# Autodesk Inventor assembly: Quad Cart
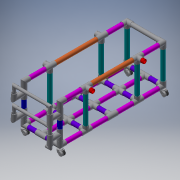
[picture p0: Inventor's stored thumbnail of the model, 180x180]
Saved by Autodesk Inventor 2018 (Build 220112000, 112)
## iProperties
Created: 2017-11-03
Part Number: Quad Cart
Document SubType Name: Assembly
Designer: owner
Author: owner
## Documents named in this file (29)
- Z:\The Pickle\Final Carts\Quad Cart.iam
- Z:\The Pickle\Inventor Pipe Parts\1.5 3-way 90.ipt
- Z:\The Pickle\Inventor Pipe Parts\Quad Pipes\1.5 pipe - 1.ipt
- Z:\The Pickle\Inventor Pipe Parts\Quad Pipes\1.5 pipe - 2.ipt
- Z:\The Pickle\Inventor Pipe Parts\1.5 Tee.ipt
- Z:\The Pickle\Inventor Pipe Parts\1.5 Tee 4-way.ipt
- Z:\The Pickle\Inventor Pipe Parts\Quad Pipes\1.5 pipe - 7.ipt
- Z:\The Pickle\Inventor Pipe Parts\Quad Pipes\1.5 pipe - 3.ipt
- Z:\The Pickle\Inventor Pipe Parts\1.5 cross.ipt
- Z:\The Pickle\Inventor Pipe Parts\Quad Pipes\1.5 pipe - 6.ipt
- Z:\The Pickle\Inventor Pipe Parts\1.5 90.ipt
- Z:\The Pickle\Inventor Pipe Parts\Quad Pipes\1.5 pipe - 4.ipt
- Z:\The Pickle\Inventor Pipe Parts\1.5 Tee 4-way_MIR.ipt
- Z:\The Pickle\Inventor Pipe Parts\Quad Pipes\1.5 pipe - 1_MIR.ipt
- Z:\The Pickle\Inventor Pipe Parts\Quad Pipes\1.5 pipe - 2_MIR.ipt
- Z:\The Pickle\Inventor Pipe Parts\Quad Pipes\1.5 pipe - 3_MIR.ipt
- Z:\The Pickle\Inventor Pipe Parts\1.5 Tee_MIR.ipt
- Z:\The Pickle\Inventor Pipe Parts\1.5 3-way 90_MIR.ipt
- Z:\The Pickle\Inventor Pipe Parts\Quad Pipes\1.5 pipe - 4_MIR.ipt
- Z:\The Pickle\Inventor Pipe Parts\Quad Pipes\1.5 pipe - 2_MIR_MIR.ipt
- Z:\The Pickle\Inventor Pipe Parts\Quad Pipes\1.5 pipe - 5.ipt
- Z:\The Pickle\Inventor Pipe Parts\Quad Pipes\1 pipe - 1.ipt
- Z:\The Pickle\Inventor Pipe Parts\Quad Pipes\1 pipe - 2.ipt
- Z:\The Pickle\Inventor Pipe Parts\Quad Pipes\1 pipe - 3.ipt
- Z:\The Pickle\Inventor Pipe Parts\Quad Pipes\1 pipe - 4.ipt
- Z:\The Pickle\Inventor Pipe Parts\1 90.ipt
- Z:\The Pickle\Inventor Pipe Parts\1 tee.ipt
- Z:\The Pickle\Inventor Pipe Parts\Wheel Part.ipt
- Z:\The Pickle\Inventor Pipe Parts\NUT.ipt
## Components (97 placed, 28 different names)
1. 1.5 3-way 90:1 — Insert:1, Insert:41, Insert:106, Insert:113, Flush:1, Insert:120
2. 1.5 pipe - 1:1 — Insert:41, Insert:42
3. 1.5 pipe - 2:1 — Insert:1, Insert:22
4. 1.5 Tee:2 — Insert:42, Insert:43, Insert:45
5. 1.5 Tee 4-way:1 — Insert:22, Insert:24, Insert:35, Insert:60
6. 1.5 Tee:3 — Insert:4, Insert:6, Insert:107
7. 1.5 pipe - 1:2 — Insert:43, Insert:44
8. 1.5 pipe - 1:3 — Insert:59, Insert:60
9. 1.5 pipe - 7:1 — Insert:6, Insert:7
10. 1.5 pipe - 2:2 — Insert:45, Insert:46
11. 1.5 pipe - 2:3 — Insert:24, Insert:27
12. 1.5 pipe - 3:1 — Insert:35, Insert:127
13. 1.5 3-way 90:2 — Insert:44, Insert:71, Insert:108, Insert:114, Insert:119
14. 1.5 Tee:4 — Insert:27, Insert:28, Insert:58
15. 1.5 Tee:5 — Insert:5
16. 1.5 Tee:6 — Insert:7, Insert:8, Insert:105
17. 1.5 cross:1 — Insert:46, Insert:47, Insert:59, Insert:61
18. 1.5 pipe - 6:1 — Insert:4, Insert:5
19. 1.5 pipe - 6:2 — Insert:8, Insert:9
20. 1.5 pipe - 6:3 — Insert:14, Insert:15
21. 1.5 pipe - 6:4 — Insert:18, Insert:19
22. 1.5 pipe - 7:2 — Insert:16, Insert:17
23. 1.5 Tee:8 — Insert:14, Insert:16, Insert:109
24. 1.5 Tee:9 — Insert:17, Insert:18, Insert:103
25. 1.5 90:1 — Insert:15
26. 1.5 90:2 — Insert:19
27. 1.5 90:3 — Insert:23, Insert:104
28. 1.5 Tee:10 — Insert:9, Insert:112
29. 1.5 90:4 — Insert:88, Insert:102
30. 1.5 cross:2 — Insert:48, Insert:49, Insert:57, Insert:62
31. 1.5 cross:3 — Insert:50, Insert:51, Insert:55, Insert:63
32. 1.5 Tee:11 — Insert:52, Insert:53, Insert:64
33. 1.5 pipe - 2:4 — Insert:47, Insert:48
34. 1.5 pipe - 2:5 — Insert:49, Insert:50
35. 1.5 pipe - 2:6 — Insert:51, Insert:52
36. 1.5 pipe - 2:7 — Insert:28, Insert:29
37. 1.5 pipe - 2:8 — Insert:30, Insert:31
38. 1.5 Tee 4-way:2 — Insert:29, Insert:30, Insert:37, Insert:56
39. 1.5 3-way 90:3 — Insert:31, Insert:39, Insert:54, Insert:115, Insert:117
40. 1.5 pipe - 1:4 — Insert:57, Insert:58
41. 1.5 pipe - 1:5 — Insert:53, Insert:54
42. 1.5 pipe - 1:6 — Insert:55, Insert:56
43. 1.5 pipe - 3:2 — Insert:39, Insert:40
44. 1.5 pipe - 3:3 — Insert:37, Insert:130
45. 1.5 pipe - 2:9 — Insert:23, Insert:128
46. 1.5 pipe - 2:10 — Insert:34, Insert:132
47. 1.5 3-way 90:4 — Insert:34, Insert:40, Insert:89
48. 1.5 pipe - 4:1 — Insert:129, Insert:131
49. 1.5 Tee 4-way_MIR:1 — Insert:68, Insert:69, Insert:70, Insert:73
50. 1.5 pipe - 1_MIR:1 — Insert:61, Insert:68
51. 1.5 pipe - 2_MIR:1 — Insert:72, Insert:73
52. 1.5 pipe - 3_MIR:1 — Insert:69, Insert:121
53. 1.5 Tee_MIR:1 — Insert:67, Insert:72, Insert:75
54. 1.5 pipe - 2_MIR:2 — Insert:74, Insert:75
55. 1.5 pipe - 2_MIR:3 — Insert:76, Insert:77
56. 1.5 Tee 4-way_MIR:2 — Insert:66, Insert:74, Insert:77, Insert:83
57. 1.5 3-way 90_MIR:1 — Insert:65, Insert:76, Insert:84, Insert:116, Insert:118
58. 1.5 pipe - 1_MIR:2 — Insert:62, Insert:67
59. 1.5 pipe - 1_MIR:3 — Insert:63, Insert:66
60. 1.5 pipe - 1_MIR:4 — Insert:64, Insert:65
61. 1.5 pipe - 3_MIR:2 — Insert:84, Insert:85
62. 1.5 pipe - 3_MIR:3 — Insert:83, Insert:124
63. 1.5 pipe - 2_MIR:4 — Insert:88, Insert:122
64. 1.5 pipe - 2_MIR:5 — Insert:82, Insert:126
65. 1.5 3-way 90_MIR:2 — Insert:82, Insert:85, Insert:90
66. 1.5 pipe - 4_MIR:1 — Insert:123, Insert:125
67. 1.5 pipe - 2_MIR_MIR:1 — Insert:70, Insert:71
68. 1.5 pipe - 5:1 — Insert:89, Insert:90
69. 1 pipe - 1:1 — Insert:100
70. 1 pipe - 1:2 — Insert:98
71. 1 pipe - 2:1 — Insert:110, Insert:111, Insert:112
72. 1 pipe - 3:1 — Insert:91, Insert:92
73. 1 pipe - 4:1 — Insert:96, Insert:97
74. 1 90:1 — Insert:91
75. 1 90:2 — Insert:96, Insert:110
76. 1 90:3 — Insert:97, Insert:98
77. 1 90:4 — Insert:99, Insert:100
78. 1 tee:1 — Insert:92, Insert:95, Insert:111
79. 1 pipe - 4:2 — Insert:95, Insert:99
80. 1.5 pipe - 6:5 — Insert:102, Insert:103
81. 1.5 pipe - 6:6 — Insert:108, Insert:109
82. 1.5 pipe - 6:7 — Insert:106, Insert:107
83. 1.5 pipe - 6:8 — Insert:104, Insert:105
84. Wheel Part:1 — Insert:114
85. Wheel Part:2 — Insert:115
86. Wheel Part:3 — Insert:116
87. Wheel Part:4 — Insert:113
88. NUT:1 — Insert:120
89. NUT:2 — Insert:119
90. NUT:3 — Insert:118
91. NUT:4 — Insert:117
92. 1.5 Tee 4-way:3 — Insert:121, Insert:122, Insert:123
93. 1.5 Tee 4-way:4 — Insert:124, Insert:125, Insert:126, Angle:2, Tangent:1
94. 1.5 Tee 4-way:5 — Insert:130, Insert:131, Insert:132, Insert:134, Angle:1
95. 1.5 Tee 4-way:6 — Insert:127, Insert:128, Insert:129, Insert:133
96. 1.5 pipe - 6:9 — Insert:133
97. 1.5 pipe - 6:10 — Insert:134
## Relationships (115: Insert 111, Angle 2, Flush 1, Tangent 1)
- Insert:1: 1.5 3-way 90:1 ↔ 1.5 pipe - 2:1
- Insert:4: 1.5 Tee:3 ↔ 1.5 pipe - 6:1
- Insert:5: 1.5 Tee:5 ↔ 1.5 pipe - 6:1
- Insert:6: 1.5 Tee:3 ↔ 1.5 pipe - 7:1
- Insert:7: 1.5 pipe - 7:1 ↔ 1.5 Tee:6
- Insert:8: 1.5 Tee:6 ↔ 1.5 pipe - 6:2
- Insert:9: 1.5 pipe - 6:2 ↔ 1.5 Tee:10
- Insert:14: 1.5 pipe - 6:3 ↔ 1.5 Tee:8
- Insert:15: 1.5 pipe - 6:3 ↔ 1.5 90:1
- Insert:16: 1.5 pipe - 7:2 ↔ 1.5 Tee:8
- Insert:17: 1.5 pipe - 7:2 ↔ 1.5 Tee:9
- Insert:18: 1.5 pipe - 6:4 ↔ 1.5 Tee:9
- Insert:19: 1.5 pipe - 6:4 ↔ 1.5 90:2
- Insert:22: 1.5 pipe - 2:1 ↔ 1.5 Tee 4-way:1
- Insert:23: 1.5 90:3 ↔ 1.5 pipe - 2:9
- Insert:24: 1.5 Tee 4-way:1 ↔ 1.5 pipe - 2:3
- Insert:27: 1.5 pipe - 2:3 ↔ 1.5 Tee:4
- Insert:28: 1.5 Tee:4 ↔ 1.5 pipe - 2:7
- Insert:29: 1.5 pipe - 2:7 ↔ 1.5 Tee 4-way:2
- Insert:30: 1.5 pipe - 2:8 ↔ 1.5 Tee 4-way:2
- Insert:31: 1.5 pipe - 2:8 ↔ 1.5 3-way 90:3
- Insert:34: 1.5 pipe - 2:10 ↔ 1.5 3-way 90:4
- Insert:35: 1.5 Tee 4-way:1 ↔ 1.5 pipe - 3:1
- Insert:37: 1.5 Tee 4-way:2 ↔ 1.5 pipe - 3:3
- Insert:39: 1.5 3-way 90:3 ↔ 1.5 pipe - 3:2
- Insert:40: 1.5 pipe - 3:2 ↔ 1.5 3-way 90:4
- Insert:41: 1.5 3-way 90:1 ↔ 1.5 pipe - 1:1
- Insert:42: 1.5 pipe - 1:1 ↔ 1.5 Tee:2
- Insert:43: 1.5 Tee:2 ↔ 1.5 pipe - 1:2
- Insert:44: 1.5 pipe - 1:2 ↔ 1.5 3-way 90:2
- Insert:45: 1.5 Tee:2 ↔ 1.5 pipe - 2:2
- Insert:46: 1.5 pipe - 2:2 ↔ 1.5 cross:1
- Insert:47: 1.5 cross:1 ↔ 1.5 pipe - 2:4
- Insert:48: 1.5 cross:2 ↔ 1.5 pipe - 2:4
- Insert:49: 1.5 cross:2 ↔ 1.5 pipe - 2:5
- Insert:50: 1.5 cross:3 ↔ 1.5 pipe - 2:5
- Insert:51: 1.5 cross:3 ↔ 1.5 pipe - 2:6
- Insert:52: 1.5 Tee:11 ↔ 1.5 pipe - 2:6
- Insert:53: 1.5 Tee:11 ↔ 1.5 pipe - 1:5
- Insert:54: 1.5 3-way 90:3 ↔ 1.5 pipe - 1:5
- Insert:55: 1.5 cross:3 ↔ 1.5 pipe - 1:6
- Insert:56: 1.5 Tee 4-way:2 ↔ 1.5 pipe - 1:6
- Insert:57: 1.5 cross:2 ↔ 1.5 pipe - 1:4
- Insert:58: 1.5 Tee:4 ↔ 1.5 pipe - 1:4
- Insert:59: 1.5 pipe - 1:3 ↔ 1.5 cross:1
- Insert:60: 1.5 Tee 4-way:1 ↔ 1.5 pipe - 1:3
- Insert:61: 1.5 cross:1 ↔ 1.5 pipe - 1_MIR:1
- Insert:62: 1.5 cross:2 ↔ 1.5 pipe - 1_MIR:2
- Insert:63: 1.5 cross:3 ↔ 1.5 pipe - 1_MIR:3
- Insert:64: 1.5 Tee:11 ↔ 1.5 pipe - 1_MIR:4
- Insert:65: 1.5 3-way 90_MIR:1 ↔ 1.5 pipe - 1_MIR:4
- Insert:66: 1.5 Tee 4-way_MIR:2 ↔ 1.5 pipe - 1_MIR:3
- Insert:67: 1.5 Tee_MIR:1 ↔ 1.5 pipe - 1_MIR:2
- Insert:68: 1.5 Tee 4-way_MIR:1 ↔ 1.5 pipe - 1_MIR:1
- Insert:69: 1.5 Tee 4-way_MIR:1 ↔ 1.5 pipe - 3_MIR:1
- Insert:70: 1.5 Tee 4-way_MIR:1 ↔ 1.5 pipe - 2_MIR_MIR:1
- Insert:71: 1.5 3-way 90:2 ↔ 1.5 pipe - 2_MIR_MIR:1
- Insert:72: 1.5 pipe - 2_MIR:1 ↔ 1.5 Tee_MIR:1
- Insert:73: 1.5 Tee 4-way_MIR:1 ↔ 1.5 pipe - 2_MIR:1
- Insert:74: 1.5 pipe - 2_MIR:2 ↔ 1.5 Tee 4-way_MIR:2
- Insert:75: 1.5 Tee_MIR:1 ↔ 1.5 pipe - 2_MIR:2
- Insert:76: 1.5 pipe - 2_MIR:3 ↔ 1.5 3-way 90_MIR:1
- Insert:77: 1.5 pipe - 2_MIR:3 ↔ 1.5 Tee 4-way_MIR:2
- Insert:82: 1.5 pipe - 2_MIR:5 ↔ 1.5 3-way 90_MIR:2
- Insert:83: 1.5 Tee 4-way_MIR:2 ↔ 1.5 pipe - 3_MIR:3
- Insert:84: 1.5 3-way 90_MIR:1 ↔ 1.5 pipe - 3_MIR:2
- Insert:85: 1.5 pipe - 3_MIR:2 ↔ 1.5 3-way 90_MIR:2
- Insert:88: 1.5 90:4 ↔ 1.5 pipe - 2_MIR:4
- Insert:89: 1.5 3-way 90:4 ↔ 1.5 pipe - 5:1
- Insert:90: 1.5 3-way 90_MIR:2 ↔ 1.5 pipe - 5:1
- Insert:91: 1 pipe - 3:1 ↔ 1 90:1
- Insert:92: 1 pipe - 3:1 ↔ 1 tee:1
- Insert:95: 1 tee:1 ↔ 1 pipe - 4:2
- Insert:96: 1 pipe - 4:1 ↔ 1 90:2
- Insert:97: 1 pipe - 4:1 ↔ 1 90:3
- Insert:98: 1 pipe - 1:2 ↔ 1 90:3
- Insert:99: 1 90:4 ↔ 1 pipe - 4:2
- Insert:100: 1 pipe - 1:1 ↔ 1 90:4
- Insert:102: 1.5 90:4 ↔ 1.5 pipe - 6:5
- Insert:103: 1.5 Tee:9 ↔ 1.5 pipe - 6:5
- Insert:104: 1.5 90:3 ↔ 1.5 pipe - 6:8
- Insert:105: 1.5 Tee:6 ↔ 1.5 pipe - 6:8
- Insert:106: 1.5 3-way 90:1 ↔ 1.5 pipe - 6:7
- Insert:107: 1.5 Tee:3 ↔ 1.5 pipe - 6:7
- Insert:108: 1.5 3-way 90:2 ↔ 1.5 pipe - 6:6
- Insert:109: 1.5 Tee:8 ↔ 1.5 pipe - 6:6
- Insert:110: 1 pipe - 2:1 ↔ 1 90:2
- Insert:111: 1 pipe - 2:1 ↔ 1 tee:1
- Insert:112: 1.5 Tee:10 ↔ 1 pipe - 2:1
- Insert:113 (88.9 mm): 1.5 3-way 90:1 ↔ Wheel Part:4
- Insert:114 (88.9 mm): 1.5 3-way 90:2 ↔ Wheel Part:1
- Insert:115 (88.9 mm): 1.5 3-way 90:3 ↔ Wheel Part:2
- Flush:1 (-88.9 mm): 1.5 3-way 90:1
- Insert:116 (88.9 mm): 1.5 3-way 90_MIR:1 ↔ Wheel Part:3
- Insert:117 (-78.74 mm): 1.5 3-way 90:3 ↔ NUT:4
- Insert:118 (78.74 mm): 1.5 3-way 90_MIR:1 ↔ NUT:3
- Insert:119 (78.74 mm): 1.5 3-way 90:2 ↔ NUT:2
- Insert:120 (78.74 mm): 1.5 3-way 90:1 ↔ NUT:1
- Insert:121: 1.5 pipe - 3_MIR:1 ↔ 1.5 Tee 4-way:3
- Insert:122: 1.5 pipe - 2_MIR:4 ↔ 1.5 Tee 4-way:3
- Insert:123: 1.5 pipe - 4_MIR:1 ↔ 1.5 Tee 4-way:3
- Insert:124: 1.5 pipe - 3_MIR:3 ↔ 1.5 Tee 4-way:4
- Insert:125: 1.5 pipe - 4_MIR:1 ↔ 1.5 Tee 4-way:4
- Insert:126: 1.5 pipe - 2_MIR:5 ↔ 1.5 Tee 4-way:4
- Insert:127: 1.5 pipe - 3:1 ↔ 1.5 Tee 4-way:6
- Insert:128: 1.5 pipe - 2:9 ↔ 1.5 Tee 4-way:6
- Insert:129: 1.5 pipe - 4:1 ↔ 1.5 Tee 4-way:6
- Insert:130: 1.5 pipe - 3:3 ↔ 1.5 Tee 4-way:5
- Insert:131: 1.5 pipe - 4:1 ↔ 1.5 Tee 4-way:5
- Insert:132: 1.5 pipe - 2:10 ↔ 1.5 Tee 4-way:5
- Insert:133: 1.5 Tee 4-way:6 ↔ 1.5 pipe - 6:9
- Insert:134: 1.5 Tee 4-way:5 ↔ 1.5 pipe - 6:10
- Angle:1 (0 deg): 1.5 Tee 4-way:5
- Angle:2 (0 deg): 1.5 Tee 4-way:4
- Tangent:1: 1.5 Tee 4-way:4
